# Autodesk Inventor assembly: RSX Assembly2
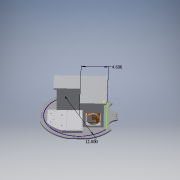
[picture p0: Inventor's stored thumbnail of the model, 180x180]
Saved by Autodesk Inventor 2016 (Build 200138000, 138)
## iProperties
Created: 2016-10-28
Part Number: RSX Assembly2
Document SubType Name: Assembly
Designer: eschr_000
Author: eschr_000
## Documents named in this file (9)
- F:\CADD\RSX structure separate walls\RSX Assembly2.iam
- C:\Users\Ethan\Desktop\RSX Assembly\RSX Structure.ipt
- C:\Users\Ethan\Desktop\RSX Assembly\VR Camera.ipt
- C:\Users\Ethan\Desktop\RSX Assembly\VR Camera Dome.ipt
- C:\Users\Ethan\Desktop\RSX Assembly\RSX Deck.ipt
- F:\CADD\RSX Assembly\Hermes Cube.iam
- C:\Users\Ethan\Desktop\RSX Assembly\0.25 Standoff.ipt
- F:\CADD\RSX structure separate walls\RSX top.ipt
- F:\star.ipt
## Components (11 placed, 8 different names)
1. RSX Structure:1 — Flush:1, Mate:13, Mate:25, Mate:26, Mate:34, Mate:35, Mate:37, Mate:38, Mate:39, Mate:40, Mate:41, Mate:42, Mate:43, Mate:44, Mate:49, Mate:50, Rigid:1
2. VR Camera:1 — Flush:1, Mate:13, Mate:14, Mate:15, Mate:25
3. VR Camera Dome:1 — Mate:14, Mate:15
4. RSX Deck:1 — Mate:26, Mate:33, Mate:36
5. Hermes Cube:1 [sub-assembly] — Mate:34, Mate:35, Mate:45
6. 0.25 Standoff:1 — Mate:40, Mate:41, Mate:45
7. 0.25 Standoff:2 — Mate:39, Mate:42
8. 0.25 Standoff:3 — Mate:37, Mate:44
9. 0.25 Standoff:4 — Mate:38, Mate:43
10. RSX top:1 — Rigid:1
11. star:1 — Mate:49, Mate:50
## Relationships (22: Mate 20, Flush 1, WeldJoint 1)
- Flush:1: RSX Structure:1 ↔ VR Camera:1
- Mate:13 (28 mm): RSX Structure:1 ↔ VR Camera:1
- Mate:14: VR Camera:1 ↔ VR Camera Dome:1
- Mate:15: VR Camera:1 ↔ VR Camera Dome:1
- Mate:25 (38.1 mm): RSX Structure:1 ↔ VR Camera:1
- Mate:26: RSX Structure:1 ↔ RSX Deck:1
- Mate:33: RSX Deck:1
- Mate:34: RSX Structure:1 ↔ Hermes Cube:1
- Mate:35 (5.475 mm): RSX Structure:1 ↔ Hermes Cube:1
- Mate:36: RSX Deck:1
- Mate:37: RSX Structure:1 ↔ 0.25 Standoff:3
- Mate:38: RSX Structure:1 ↔ 0.25 Standoff:4
- Mate:39: RSX Structure:1 ↔ 0.25 Standoff:2
- Mate:40: RSX Structure:1 ↔ 0.25 Standoff:1
- Mate:41: RSX Structure:1 ↔ 0.25 Standoff:1
- Mate:42: RSX Structure:1 ↔ 0.25 Standoff:2
- Mate:43: RSX Structure:1 ↔ 0.25 Standoff:4
- Mate:44: RSX Structure:1 ↔ 0.25 Standoff:3
- Mate:45: Hermes Cube:1 ↔ 0.25 Standoff:1
- Mate:49: RSX Structure:1 ↔ star:1
- Mate:50: RSX Structure:1 ↔ star:1
- Rigid:1 [WeldJoint] (12.7 mm): RSX Structure:1 ↔ RSX top:1
